# Autodesk Inventor assembly: DriveBase
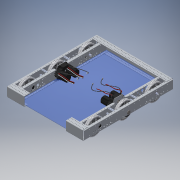
[picture p0: Inventor's stored thumbnail of the model, 180x180]
Saved by Autodesk Inventor 2019 (Build 230136000, 136)
## iProperties
Created: 2020-01-13
Part Number: DriveBase
Document SubType Name: Assembly
Designer: james
Author: james
## Documents named in this file (5)
- F:\JimsRobot\FIRSTRobots\Design\JimsCHS2020FRC\DriveBase.iam
- F:\JimsRobot\FIRSTRobots\Design\JimsCHS2020FRC\SideBeam.iam
- F:\JimsRobot\FIRSTRobots\Design\JimsCHS2020FRC\BackBar.ipt
- F:\JimsRobot\FIRSTRobots\Design\JimsCHS2020FRC\FrontBar.ipt
- F:\JimsRobot\FIRSTRobots\Design\JimsCHS2020FRC\BellyPan.ipt
## Components (6 placed, 4 different names)
1. SideBeam:1 [sub-assembly] — Mate:5, Mate:8, Mate:9, Mate:10, Mate:13, Mate:15, Mate:16
2. SideBeam:2 [sub-assembly] — Mate:1, Mate:2, Mate:3, Mate:7, Mate:11, Mate:12
3. BackBar:1 — Mate:1, Mate:2, Mate:3, Mate:5, Mate:14, Mate:16
4. FrontBar:1 — Mate:8, Mate:9, Mate:10
5. FrontBar:2 — Mate:7, Mate:11, Mate:12
6. BellyPan:1 — Mate:13, Mate:14, Mate:15
## Relationships (14: Mate 14)
- Mate:1: SideBeam:2 ↔ BackBar:1
- Mate:2: SideBeam:2 ↔ BackBar:1
- Mate:3: SideBeam:2 ↔ BackBar:1
- Mate:5: SideBeam:1 ↔ BackBar:1
- Mate:7: SideBeam:2 ↔ FrontBar:2
- Mate:8: SideBeam:1 ↔ FrontBar:1
- Mate:9: SideBeam:1 ↔ FrontBar:1
- Mate:10: SideBeam:1 ↔ FrontBar:1
- Mate:11: SideBeam:2 ↔ FrontBar:2
- Mate:12: SideBeam:2 ↔ FrontBar:2
- Mate:13: SideBeam:1 ↔ BellyPan:1
- Mate:14: BackBar:1 ↔ BellyPan:1
- Mate:15: SideBeam:1 ↔ BellyPan:1
- Mate:16: SideBeam:1 ↔ BackBar:1
